# Autodesk Inventor assembly: stand_cam
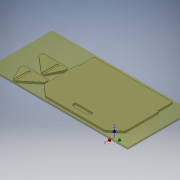
[picture p0: Inventor's stored thumbnail of the model, 180x180]
Saved by Autodesk Inventor 2016 (Build 200138000, 138)
## iProperties
Created: 2016-10-18
Part Number: stand_cam
Document SubType Name: Assembly
Designer: rawrdong
Author: rawrdong
## Documents named in this file (4)
- C:\Users\rawrdong\Box Sync\0_GradSchoolResearch\00_projects\0_AirParticleCounter\NEW_SHIT\NEBULIZER\stand_cam.iam
- C:\Users\rawrdong\Box Sync\0_GradSchoolResearch\00_projects\0_AirParticleCounter\NEW_SHIT\NEBULIZER\back_1.ipt
- C:\Users\rawrdong\Box Sync\0_GradSchoolResearch\00_projects\0_AirParticleCounter\NEW_SHIT\NEBULIZER\foot_1.ipt
- C:\Users\rawrdong\Box Sync\0_GradSchoolResearch\00_projects\0_AirParticleCounter\NEW_SHIT\NEBULIZER\foot_flipped_1.ipt
## Components (3 placed, 3 different names)
1. back_1:1 — Flush:1, Flush:2
2. foot_1:1 — Flush:1
3. foot_flipped_1:1 — Flush:2
## Relationships (2: Flush 2)
- Flush:1: back_1:1 ↔ foot_1:1
- Flush:2: back_1:1 ↔ foot_flipped_1:1
